# Autodesk Inventor assembly: rbc support
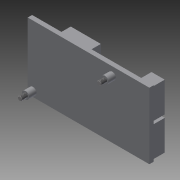
[picture p0: Inventor's stored thumbnail of the model, 180x180]
Saved by Autodesk Inventor 2015 (Build 190159000, 159)
## iProperties
Created: 2015-05-04
Part Number: rbc support
Document SubType Name: Assembly
Designer: Kuba
Author: Kuba
## Documents named in this file (4)
- C:\Users\Kuba\Dysk Google\synergia\Synergolf\model\GOLF\rbc support\rbc support.iam
- C:\Users\Kuba\Dysk Google\synergia\Synergolf\model\GOLF\RBC4242.ipt
- C:\Users\Kuba\Dysk Google\synergia\Synergolf\model\GOLF\ContentCenter\pl-PL\DIN 912\DIN 912 - M3 x 0,5 x 12 x 10,75.ipt
- C:\Users\Kuba\Dysk Google\synergia\Synergolf\model\GOLF\batt support\dystans rbc.ipt
## Components (5 placed, 3 different names)
1. RBC4242:1 — Zestawiający:3, Zestawiający:4, Zestawiający:5, Zestawiający:6, Wstaw:1, Wstaw:2
2. DIN 912 - zastąpiona przez DIN EN ISO 4762 M3 x 12:1 — Zestawiający:3, Zestawiający:4
3. DIN 912 - zastąpiona przez DIN EN ISO 4762 M3 x 12:2 — Zestawiający:5, Zestawiający:6
4. dystans rbc:1 — Wstaw:1
5. dystans rbc:2 — Wstaw:2
## Relationships (6: Mate 4, Insert 2)
- Zestawiający:3 [Mate]: RBC4242:1 ↔ DIN 912 - zastąpiona przez DIN EN ISO 4762 M3 x 12:1
- Zestawiający:4 [Mate]: RBC4242:1 ↔ DIN 912 - zastąpiona przez DIN EN ISO 4762 M3 x 12:1
- Zestawiający:5 [Mate]: RBC4242:1 ↔ DIN 912 - zastąpiona przez DIN EN ISO 4762 M3 x 12:2
- Zestawiający:6 [Mate]: RBC4242:1 ↔ DIN 912 - zastąpiona przez DIN EN ISO 4762 M3 x 12:2
- Wstaw:1 [Insert]: RBC4242:1 ↔ dystans rbc:1
- Wstaw:2 [Insert]: RBC4242:1 ↔ dystans rbc:2
